# Autodesk Inventor assembly: Motor Driver V1.4
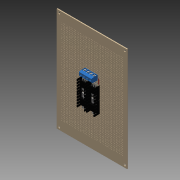
[picture p0: Inventor's stored thumbnail of the model, 180x180]
Saved by Autodesk Inventor 2015 (Build 190159000, 159)
## iProperties
Created: 2016-01-20
Part Number: Motor Driver V1.4
Document SubType Name: Assembly
Designer: Kyle
Author: Kyle
## Documents named in this file (18)
- C:\Users\Kyle\Documents\Project documentation\Motor driver\V1.4\CAD\Motor Driver V1.4.iam
- C:\Users\Kyle\Documents\Project documentation\Motor driver\V1.4\CAD\40x55 PC Board.ipt
- C:\Users\Kyle\Documents\Project documentation\Motor driver\V1.4\CAD\TO-220 Heatsink.ipt
- C:\Users\Kyle\Documents\Project documentation\Motor driver\V1.4\CAD\TO-220 Thermal Film.ipt
- C:\Users\Kyle\Documents\Project documentation\Motor driver\V1.4\CAD\TO-220 Transistor.iam
- C:\Users\Kyle\Documents\Project documentation\Motor driver\V1.4\CAD\6-32 14'' Screw.ipt
- C:\Users\Kyle\Documents\Project documentation\Motor driver\V1.4\CAD\6-32 Nut.ipt
- C:\Users\Kyle\Documents\Project documentation\Motor driver\V1.4\CAD\s470 Resistor.ipt
- C:\Users\Kyle\Documents\Project documentation\Motor driver\V1.4\CAD\Solder Joint.ipt
- C:\Users\Kyle\Documents\Project documentation\Motor driver\V1.4\CAD\sTLP152 Optocoupler.ipt
- C:\Users\Kyle\Documents\Project documentation\Motor driver\V1.4\CAD\s1k Resistor.ipt
- C:\Users\Kyle\Documents\Project documentation\Motor driver\V1.4\CAD\74LVC2G14 Dual Inverter.ipt
- C:\Users\Kyle\Documents\Project documentation\Motor driver\V1.4\CAD\s174 Resistor.ipt
- C:\Users\Kyle\Documents\Project documentation\Motor driver\V1.4\CAD\s74LVC2G08 Dual AND.ipt
- C:\Users\Kyle\Documents\Project documentation\Motor driver\V1.4\CAD\1x2 Terminal Block.iam
- C:\Users\Kyle\Documents\Project documentation\Motor driver\V1.4\CAD\s1uF Capacitor.ipt
- C:\Users\Kyle\Documents\Project documentation\Motor driver\V1.4\CAD\s20A 60V Diode.ipt
- C:\Users\Kyle\Documents\Project documentation\Motor driver\V1.4\CAD\Wire 3.ipt
## Components (95 placed, 17 different names)
1. 40x55 PC Board:1 — Mate:1, Mate:2, Mate:3, Mate:4, Mate:5, Angle:1, Mate:6, Angle:2, Angle:3, Mate:7, Mate:8, Mate:18, Mate:19, Mate:21, Mate:22, Mate:24, Mate:25, Mate:27, Mate:28, Mate:29, Mate:31, Mate:33, Mate:35, Mate:37, Mate:39, Mate:41, Mate:43, Mate:45, Angle:8, Mate:46, Mate:47, Mate:48, Mate:49, Angle:9, Mate:50, Mate:51, Mate:52, Mate:53, Mate:55, Mate:56, Mate:58, Mate:59, Mate:61, Mate:62, Mate:64, Mate:65, Mate:67, Mate:68, Mate:70, Mate:71, Mate:73, Mate:74, Mate:75, Mate:76, Mate:77, Mate:79, Mate:80, Mate:83, Mate:86, Mate:91, Mate:92, Mate:95, Mate:99, Mate:101, Mate:102, Mate:103, Mate:105, Mate:106, Angle:10, Flush:4, Mate:107, Mate:108, Mate:109, Flush:5, Mate:110, Mate:112, Mate:113, Flush:6, Flush:7, Flush:8, Flush:9, Mate:115, Mate:116, Mate:117, Mate:118, Mate:119, Mate:120, Flush:10, Flush:11, Flush:12, Flush:13, Mate:121, Mate:122, Mate:123, Mate:125, Mate:126, Mate:127, Mate:129, Mate:130, Mate:131, Mate:133, Mate:134, Mate:135, Mate:136, Mate:137, Mate:138, Mate:139, Mate:141, Mate:142, Mate:144, Mate:145, Mate:146, Mate:147, Mate:148, Mate:154, Mate:155, Mate:156, Mate:157, Flush:14, Flush:15, Mate:160, Mate:161, Mate:162, Mate:163, Mate:164, Mate:165, Mate:166, Mate:168, Mate:170, Mate:172, Mate:174, Mate:176, Mate:178, Mate:180, Mate:181, Mate:182, Mate:183, Mate:184, Mate:187, Mate:188, Mate:189, Mate:191, Angle:11, Mate:192, Mate:193, Mate:194, Angle:12, Angle:13, Flush:19, Flush:20, Flush:21, Mate:207, Angle:14, Mate:208, Mate:209, Mate:211, Mate:212, Mate:213, Mate:215, Mate:217, Mate:219, Mate:220, Mate:221, Mate:222, Mate:223, Mate:224, Mate:225, Mate:226, Mate:227, Mate:230, Mate:231, Mate:232, Mate:233, Mate:234, Mate:235, Mate:236, Mate:237, Mate:238, Mate:239, Mate:240, Angle:15, Tangent:1, Mate:241, Mate:242, Mate:243, Mate:244, Mate:245, Mate:247, Mate:251, Mate:252, Mate:253, Mate:254, Mate:255, Mate:256, Mate:257, Mate:259, Mate:261, Mate:263, Mate:265, Mate:267, Mate:269
2. TO-220 Heatsink:1 — Mate:1, Angle:3, Flush:3, Mate:7, Mate:9, Mate:10, Angle:4
3. TO-220 Heatsink:2 — Mate:3, Flush:1, Mate:6, Flush:2, Mate:13, Mate:14, Angle:6
4. TO-220 Heatsink:3 — Mate:2, Angle:2, Flush:2, Mate:8, Mate:15, Mate:16, Angle:7
5. TO-220 Heatsink:4 — Mate:4, Mate:5, Flush:1, Angle:1, Flush:3, Mate:11, Angle:5, Mate:12
6. TO-220 Thermal Film:1 — Mate:13, Mate:14, Angle:6, Mate:23
7. TO-220 Thermal Film:2 — Mate:15, Mate:16, Angle:7, Mate:26
8. TO-220 Thermal Film:3 — Mate:9, Mate:10, Angle:4, Mate:20
9. TO-220 Thermal Film:4 — Mate:11, Angle:5, Mate:12, Mate:17
10. TO-220 Transistor:1 [sub-assembly] — Mate:23, Mate:24, Mate:25, Mate:34
11. TO-220 Transistor:2 [sub-assembly] — Mate:26, Mate:27, Mate:28, Mate:30
12. TO-220 Transistor:3 [sub-assembly] — Mate:20, Mate:21, Mate:22, Mate:32
13. TO-220 Transistor:4 [sub-assembly] — Mate:17, Mate:18, Mate:19, Mate:36
14. 6-32 14'' Screw:1 — Mate:29, Mate:30, Mate:42
15. 6-32 14'' Screw:2 — Mate:31, Mate:32, Mate:38
16. 6-32 14'' Screw:3 — Mate:33, Mate:34, Mate:44
17. 6-32 14'' Screw:4 — Mate:35, Mate:36, Mate:40
18. 6-32 Nut:1 — Mate:37, Mate:38
19. 6-32 Nut:2 — Mate:39, Mate:40
20. 6-32 Nut:3 — Mate:41, Mate:42
21. 6-32 Nut:4 — Mate:43, Mate:44
22. s470 Resistor:1 — Mate:45, Angle:8, Mate:46, Mate:47
23. s470 Resistor:2 — Mate:48, Mate:49, Angle:9, Mate:50
24. Solder Joint:1 — Mate:72, Mate:73, Mate:74, Mate:111
25. Solder Joint:2 — Mate:69, Mate:70, Mate:71, Mate:72
26. Solder Joint:3 — Mate:63, Mate:64, Mate:65, Mate:66
27. Solder Joint:4 — Mate:51, Mate:52, Mate:53, Mate:54
28. Solder Joint:5 — Mate:54, Mate:55, Mate:56, Mate:57
29. Solder Joint:6 — Mate:60, Mate:61, Mate:62, Mate:63
30. Solder Joint:7 — Mate:57, Mate:58, Mate:59, Mate:60
31. Solder Joint:8 — Mate:66, Mate:67, Mate:68, Mate:69
32. Solder Joint:9 — Mate:75, Mate:76, Mate:77, Mate:78
33. Solder Joint:10 — Mate:78, Mate:79, Mate:80, Mate:81
34. Solder Joint:11 — Mate:81, Mate:83, Mate:99, Mate:100
35. Solder Joint:12 — Mate:86, Mate:100, Mate:101
36. Solder Joint:14 — Mate:95, Mate:102, Mate:103, Mate:104
37. Solder Joint:15 — Mate:91, Mate:92, Mate:104, Mate:114
38. sTLP152 Optocoupler:1 — Mate:106, Flush:6, Flush:7
39. sTLP152 Optocoupler:2 — Mate:105, Angle:10, Flush:4, Mate:107
40. s1k Resistor:1 — Mate:108, Mate:109, Flush:5
41. s1k Resistor:2 — Mate:113, Flush:8, Flush:9
42. Solder Joint:16 — Mate:110, Mate:111, Mate:112
43. Solder Joint:17 — Mate:114, Mate:115, Mate:116
44. 74LVC2G14 Dual Inverter:1 — Mate:117
45. s174 Resistor:1 — Mate:119, Flush:12, Flush:13
46. s174 Resistor:2 — Mate:118, Flush:10, Flush:11
47. s74LVC2G08 Dual AND:1 — Mate:120, Flush:14, Flush:15
48. Solder Joint:18 — Mate:121, Mate:122, Mate:123, Mate:124
49. Solder Joint:19 — Mate:124, Mate:125, Mate:126, Mate:128
50. Solder Joint:20 — Mate:127, Mate:128, Mate:129, Mate:132, Mate:167
51. Solder Joint:21 — Mate:130, Mate:131, Mate:132, Mate:150
52. Solder Joint:22 — Mate:133, Mate:134, Mate:135
53. Solder Joint:23 — Mate:136, Mate:137, Mate:138, Mate:140
54. Solder Joint:24 — Mate:139, Mate:140, Mate:141, Mate:143, Mate:185
55. Solder Joint:25 — Mate:142, Mate:143, Mate:144, Mate:159
56. Solder Joint:27 — Mate:148, Mate:149, Mate:150
57. Solder Joint:28 — Mate:145, Mate:146, Mate:147, Mate:149
58. Solder Joint:30 — Mate:157, Mate:158, Mate:159
59. Solder Joint:31 — Mate:154, Mate:155, Mate:156, Mate:158
60. Solder Joint:32 — Mate:160, Mate:167, Mate:168, Mate:169
61. Solder Joint:33 — Mate:161, Mate:169, Mate:170, Mate:171
62. Solder Joint:34 — Mate:162, Mate:171, Mate:172, Mate:173
63. Solder Joint:35 — Mate:163, Mate:173, Mate:174, Mate:175
64. Solder Joint:36 — Mate:164, Mate:175, Mate:176, Mate:177
65. Solder Joint:37 — Mate:165, Mate:177, Mate:178, Mate:179
66. Solder Joint:38 — Mate:166, Mate:179, Mate:180
67. Solder Joint:39 — Mate:181, Mate:184, Mate:185, Mate:186
68. Solder Joint:40 — Mate:182, Mate:186, Mate:187
69. Solder Joint:41 — Mate:183, Mate:188, Mate:189, Mate:210
70. 1x2 Terminal Block:1 [sub-assembly] — Mate:190, Flush:16, Flush:17, Angle:11, Mate:192, Mate:214, Mate:228
71. 1x2 Terminal Block:2 [sub-assembly] — Mate:190, Flush:16, Flush:17, Mate:191, Mate:246, Mate:258
72. s1uF Capacitor:1 — Mate:193, Angle:12, Flush:18, Flush:19, Flush:20
73. s1uF Capacitor:2 — Mate:194, Angle:13, Flush:18, Flush:21
74. s20A 60V Diode:1 — Mate:207, Angle:14
75. Solder Joint:42 — Mate:208, Mate:209, Mate:210
76. Solder Joint:43 — Mate:211, Mate:214, Mate:215, Mate:216
77. Solder Joint:44 — Mate:212, Mate:218, Mate:219
78. Solder Joint:45 — Mate:213, Mate:216, Mate:217, Mate:218
79. Solder Joint:46 — Mate:220, Mate:227, Mate:228, Mate:229
80. Solder Joint:47 — Mate:221, Mate:229, Mate:230, Mate:232
81. Solder Joint:48 — Mate:222, Mate:231, Mate:234
82. Solder Joint:49 — Mate:223, Mate:233, Mate:236
83. Solder Joint:50 — Mate:224, Mate:235, Mate:238
84. Solder Joint:51 — Mate:225, Mate:237
85. Solder Joint:52 — Mate:226, Mate:239, Mate:240
86. Wire 3:1 — Angle:15, Tangent:1, Mate:241, Mate:242, Mate:249, Mate:250
87. Solder Joint:53 — Mate:243, Mate:246, Mate:247, Mate:248
88. Solder Joint:54 — Mate:244, Mate:248, Mate:249
89. Solder Joint:55 — Mate:245, Mate:250, Mate:251
90. Solder Joint:56 — Mate:252, Mate:258, Mate:259, Mate:260
91. Solder Joint:57 — Mate:253, Mate:260, Mate:261, Mate:262
92. Solder Joint:58 — Mate:254, Mate:262, Mate:263, Mate:264
93. Solder Joint:59 — Mate:255, Mate:264, Mate:265, Mate:266
94. Solder Joint:60 — Mate:256, Mate:266, Mate:267, Mate:268
95. Solder Joint:61 — Mate:257, Mate:268, Mate:269
## Relationships (279: Mate 242, Flush 21, Angle 15, Tangent 1)
- Mate:1: 40x55 PC Board:1 ↔ TO-220 Heatsink:1
- Mate:2: 40x55 PC Board:1 ↔ TO-220 Heatsink:3
- Mate:3: 40x55 PC Board:1 ↔ TO-220 Heatsink:2
- Mate:4: 40x55 PC Board:1 ↔ TO-220 Heatsink:4
- Mate:5: 40x55 PC Board:1 ↔ TO-220 Heatsink:4
- Flush:1: TO-220 Heatsink:2 ↔ TO-220 Heatsink:4
- Angle:1 (0 deg): 40x55 PC Board:1 ↔ TO-220 Heatsink:4
- Mate:6: 40x55 PC Board:1 ↔ TO-220 Heatsink:2
- Angle:2 (0 deg): 40x55 PC Board:1 ↔ TO-220 Heatsink:3
- Angle:3 (0 deg): 40x55 PC Board:1 ↔ TO-220 Heatsink:1
- Flush:2: TO-220 Heatsink:2 ↔ TO-220 Heatsink:3
- Flush:3: TO-220 Heatsink:1 ↔ TO-220 Heatsink:4
- Mate:7: 40x55 PC Board:1 ↔ TO-220 Heatsink:1
- Mate:8: 40x55 PC Board:1 ↔ TO-220 Heatsink:3
- Mate:9: TO-220 Heatsink:1 ↔ TO-220 Thermal Film:3
- Mate:10: TO-220 Heatsink:1 ↔ TO-220 Thermal Film:3
- Angle:4 (0 deg): TO-220 Heatsink:1 ↔ TO-220 Thermal Film:3
- Mate:11: TO-220 Heatsink:4 ↔ TO-220 Thermal Film:4
- Angle:5 (0 deg): TO-220 Heatsink:4 ↔ TO-220 Thermal Film:4
- Mate:12: TO-220 Heatsink:4 ↔ TO-220 Thermal Film:4
- Mate:13: TO-220 Heatsink:2 ↔ TO-220 Thermal Film:1
- Mate:14: TO-220 Heatsink:2 ↔ TO-220 Thermal Film:1
- Angle:6 (0 deg): TO-220 Heatsink:2 ↔ TO-220 Thermal Film:1
- Mate:15: TO-220 Heatsink:3 ↔ TO-220 Thermal Film:2
- Mate:16: TO-220 Heatsink:3 ↔ TO-220 Thermal Film:2
- Angle:7 (0 deg): TO-220 Heatsink:3 ↔ TO-220 Thermal Film:2
- Mate:17: TO-220 Thermal Film:4 ↔ TO-220 Transistor:4
- Mate:18: 40x55 PC Board:1 ↔ TO-220 Transistor:4
- Mate:19: 40x55 PC Board:1 ↔ TO-220 Transistor:4
- Mate:20: TO-220 Thermal Film:3 ↔ TO-220 Transistor:3
- Mate:21: 40x55 PC Board:1 ↔ TO-220 Transistor:3
- Mate:22: 40x55 PC Board:1 ↔ TO-220 Transistor:3
- Mate:23: TO-220 Thermal Film:1 ↔ TO-220 Transistor:1
- Mate:24: 40x55 PC Board:1 ↔ TO-220 Transistor:1
- Mate:25: 40x55 PC Board:1 ↔ TO-220 Transistor:1
- Mate:26: TO-220 Thermal Film:2 ↔ TO-220 Transistor:2
- Mate:27: 40x55 PC Board:1 ↔ TO-220 Transistor:2
- Mate:28: 40x55 PC Board:1 ↔ TO-220 Transistor:2
- Mate:29: 40x55 PC Board:1 ↔ 6-32 14'' Screw:1
- Mate:30: TO-220 Transistor:2 ↔ 6-32 14'' Screw:1
- Mate:31: 40x55 PC Board:1 ↔ 6-32 14'' Screw:2
- Mate:32: TO-220 Transistor:3 ↔ 6-32 14'' Screw:2
- Mate:33: 40x55 PC Board:1 ↔ 6-32 14'' Screw:3
- Mate:34: TO-220 Transistor:1 ↔ 6-32 14'' Screw:3
- Mate:35: 40x55 PC Board:1 ↔ 6-32 14'' Screw:4
- Mate:36: TO-220 Transistor:4 ↔ 6-32 14'' Screw:4
- Mate:37: 40x55 PC Board:1 ↔ 6-32 Nut:1
- Mate:38: 6-32 14'' Screw:2 ↔ 6-32 Nut:1
- Mate:39: 40x55 PC Board:1 ↔ 6-32 Nut:2
- Mate:40: 6-32 14'' Screw:4 ↔ 6-32 Nut:2
- Mate:41: 40x55 PC Board:1 ↔ 6-32 Nut:3
- Mate:42: 6-32 14'' Screw:1 ↔ 6-32 Nut:3
- Mate:43: 40x55 PC Board:1 ↔ 6-32 Nut:4
- Mate:44: 6-32 14'' Screw:3 ↔ 6-32 Nut:4
- Mate:45: 40x55 PC Board:1 ↔ s470 Resistor:1
- Angle:8 (0 deg): 40x55 PC Board:1 ↔ s470 Resistor:1
- Mate:46 (1.016 mm): 40x55 PC Board:1 ↔ s470 Resistor:1
- Mate:47 (1.778 mm): 40x55 PC Board:1 ↔ s470 Resistor:1
- Mate:48: 40x55 PC Board:1 ↔ s470 Resistor:2
- Mate:49 (1.016 mm): 40x55 PC Board:1 ↔ s470 Resistor:2
- Angle:9 (0 deg): 40x55 PC Board:1 ↔ s470 Resistor:2
- Mate:50 (1.778 mm): 40x55 PC Board:1 ↔ s470 Resistor:2
- Mate:51: 40x55 PC Board:1 ↔ Solder Joint:4
- Mate:52: 40x55 PC Board:1 ↔ Solder Joint:4
- Mate:53: 40x55 PC Board:1 ↔ Solder Joint:4
- Mate:54: Solder Joint:4 ↔ Solder Joint:5
- Mate:55: 40x55 PC Board:1 ↔ Solder Joint:5
- Mate:56: 40x55 PC Board:1 ↔ Solder Joint:5
- Mate:57: Solder Joint:5 ↔ Solder Joint:7
- Mate:58: 40x55 PC Board:1 ↔ Solder Joint:7
- Mate:59: 40x55 PC Board:1 ↔ Solder Joint:7
- Mate:60: Solder Joint:6 ↔ Solder Joint:7
- Mate:61: 40x55 PC Board:1 ↔ Solder Joint:6
- Mate:62: 40x55 PC Board:1 ↔ Solder Joint:6
- Mate:63: Solder Joint:3 ↔ Solder Joint:6
- Mate:64: 40x55 PC Board:1 ↔ Solder Joint:3
- Mate:65: 40x55 PC Board:1 ↔ Solder Joint:3
- Mate:66: Solder Joint:3 ↔ Solder Joint:8
- Mate:67: 40x55 PC Board:1 ↔ Solder Joint:8
- Mate:68: 40x55 PC Board:1 ↔ Solder Joint:8
- Mate:69: Solder Joint:2 ↔ Solder Joint:8
- Mate:70: 40x55 PC Board:1 ↔ Solder Joint:2
- Mate:71: 40x55 PC Board:1 ↔ Solder Joint:2
- Mate:72: Solder Joint:1 ↔ Solder Joint:2
- Mate:73: 40x55 PC Board:1 ↔ Solder Joint:1
- Mate:74: 40x55 PC Board:1 ↔ Solder Joint:1
- Mate:75: 40x55 PC Board:1 ↔ Solder Joint:9
- Mate:76: 40x55 PC Board:1 ↔ Solder Joint:9
- Mate:77: 40x55 PC Board:1 ↔ Solder Joint:9
- Mate:78: Solder Joint:9 ↔ Solder Joint:10
- Mate:79: 40x55 PC Board:1 ↔ Solder Joint:10
- Mate:80: 40x55 PC Board:1 ↔ Solder Joint:10
- Mate:81: Solder Joint:10 ↔ Solder Joint:11
- Mate:83: 40x55 PC Board:1 ↔ Solder Joint:11
- Mate:86: 40x55 PC Board:1 ↔ Solder Joint:12
- Mate:91: 40x55 PC Board:1 ↔ Solder Joint:15
- Mate:92: 40x55 PC Board:1 ↔ Solder Joint:15
- Mate:95: 40x55 PC Board:1 ↔ Solder Joint:14
- Mate:99: 40x55 PC Board:1 ↔ Solder Joint:11
- Mate:100: Solder Joint:11 ↔ Solder Joint:12
- Mate:101: 40x55 PC Board:1 ↔ Solder Joint:12
- Mate:102: 40x55 PC Board:1 ↔ Solder Joint:14
- Mate:103: 40x55 PC Board:1 ↔ Solder Joint:14
- Mate:104: Solder Joint:14 ↔ Solder Joint:15
- Mate:105: 40x55 PC Board:1 ↔ sTLP152 Optocoupler:2
- Mate:106: 40x55 PC Board:1 ↔ sTLP152 Optocoupler:1
- Angle:10 (0 deg): 40x55 PC Board:1 ↔ sTLP152 Optocoupler:2
- Flush:4 (51.2572 mm): 40x55 PC Board:1 ↔ sTLP152 Optocoupler:2
- Mate:107 (0.508 mm): 40x55 PC Board:1 ↔ sTLP152 Optocoupler:2
- Mate:108: 40x55 PC Board:1 ↔ s1k Resistor:1
- Mate:109 (0.381 mm): 40x55 PC Board:1 ↔ s1k Resistor:1
- Flush:5 (49.911 mm): 40x55 PC Board:1 ↔ s1k Resistor:1
- Mate:110: 40x55 PC Board:1 ↔ Solder Joint:16
- Mate:111: Solder Joint:1 ↔ Solder Joint:16
- Mate:112: 40x55 PC Board:1 ↔ Solder Joint:16
- Mate:113: 40x55 PC Board:1 ↔ s1k Resistor:2
- Flush:6 (49.276 mm): 40x55 PC Board:1 ↔ sTLP152 Optocoupler:1
- Flush:7 (105.41 mm): 40x55 PC Board:1 ↔ sTLP152 Optocoupler:1
- Flush:8 (47.879 mm): 40x55 PC Board:1 ↔ s1k Resistor:2
- Flush:9 (111.252 mm): 40x55 PC Board:1 ↔ s1k Resistor:2
- Mate:114: Solder Joint:15 ↔ Solder Joint:17
- Mate:115: 40x55 PC Board:1 ↔ Solder Joint:17
- Mate:116: 40x55 PC Board:1 ↔ Solder Joint:17
- Mate:117: 40x55 PC Board:1 ↔ 74LVC2G14 Dual Inverter:1
- Mate:118: 40x55 PC Board:1 ↔ s174 Resistor:2
- Mate:119: 40x55 PC Board:1 ↔ s174 Resistor:1
- Mate:120: 40x55 PC Board:1 ↔ s74LVC2G08 Dual AND:1
- Flush:10 (81.026 mm): 40x55 PC Board:1 ↔ s174 Resistor:2
- Flush:11 (54.864 mm): 40x55 PC Board:1 ↔ s174 Resistor:2
- Flush:12 (59.944 mm): 40x55 PC Board:1 ↔ s174 Resistor:1
- Flush:13 (63.881 mm): 40x55 PC Board:1 ↔ s174 Resistor:1
- Mate:121: 40x55 PC Board:1 ↔ Solder Joint:18
- Mate:122: 40x55 PC Board:1 ↔ Solder Joint:18
- Mate:123: 40x55 PC Board:1 ↔ Solder Joint:18
- Mate:124: Solder Joint:18 ↔ Solder Joint:19
- Mate:125: 40x55 PC Board:1 ↔ Solder Joint:19
- Mate:126: 40x55 PC Board:1 ↔ Solder Joint:19
- Mate:127: 40x55 PC Board:1 ↔ Solder Joint:20
- Mate:128: Solder Joint:19 ↔ Solder Joint:20
- Mate:129: 40x55 PC Board:1 ↔ Solder Joint:20
- Mate:130: 40x55 PC Board:1 ↔ Solder Joint:21
- Mate:131: 40x55 PC Board:1 ↔ Solder Joint:21
- Mate:132: Solder Joint:20 ↔ Solder Joint:21
- Mate:133: 40x55 PC Board:1 ↔ Solder Joint:22
- Mate:134: 40x55 PC Board:1 ↔ Solder Joint:22
- Mate:135: 40x55 PC Board:1 ↔ Solder Joint:22
- Mate:136: 40x55 PC Board:1 ↔ Solder Joint:23
- Mate:137: 40x55 PC Board:1 ↔ Solder Joint:23
- Mate:138: 40x55 PC Board:1 ↔ Solder Joint:23
- Mate:139: 40x55 PC Board:1 ↔ Solder Joint:24
- Mate:140: Solder Joint:23 ↔ Solder Joint:24
- Mate:141: 40x55 PC Board:1 ↔ Solder Joint:24
- Mate:142: 40x55 PC Board:1 ↔ Solder Joint:25
- Mate:143: Solder Joint:24 ↔ Solder Joint:25
- Mate:144: 40x55 PC Board:1 ↔ Solder Joint:25
- Mate:145: 40x55 PC Board:1 ↔ Solder Joint:28
- Mate:146: 40x55 PC Board:1 ↔ Solder Joint:28
- Mate:147: 40x55 PC Board:1 ↔ Solder Joint:28
- Mate:148: 40x55 PC Board:1 ↔ Solder Joint:27
- Mate:149: Solder Joint:27 ↔ Solder Joint:28
- Mate:150: Solder Joint:21 ↔ Solder Joint:27
- Mate:154: 40x55 PC Board:1 ↔ Solder Joint:31
- Mate:155: 40x55 PC Board:1 ↔ Solder Joint:31
- Mate:156: 40x55 PC Board:1 ↔ Solder Joint:31
- Mate:157: 40x55 PC Board:1 ↔ Solder Joint:30
- Mate:158: Solder Joint:30 ↔ Solder Joint:31
- Mate:159: Solder Joint:25 ↔ Solder Joint:30
- Flush:14 (54.61 mm): 40x55 PC Board:1 ↔ s74LVC2G08 Dual AND:1
- Flush:15 (91.186 mm): 40x55 PC Board:1 ↔ s74LVC2G08 Dual AND:1
- Mate:160: 40x55 PC Board:1 ↔ Solder Joint:32
- Mate:161: 40x55 PC Board:1 ↔ Solder Joint:33
- Mate:162: 40x55 PC Board:1 ↔ Solder Joint:34
- Mate:163: 40x55 PC Board:1 ↔ Solder Joint:35
- Mate:164: 40x55 PC Board:1 ↔ Solder Joint:36
- Mate:165: 40x55 PC Board:1 ↔ Solder Joint:37
- Mate:166: 40x55 PC Board:1 ↔ Solder Joint:38
- Mate:167: Solder Joint:20 ↔ Solder Joint:32
- Mate:168: 40x55 PC Board:1 ↔ Solder Joint:32
- Mate:169: Solder Joint:32 ↔ Solder Joint:33
- Mate:170: 40x55 PC Board:1 ↔ Solder Joint:33
- Mate:171: Solder Joint:33 ↔ Solder Joint:34
- Mate:172: 40x55 PC Board:1 ↔ Solder Joint:34
- Mate:173: Solder Joint:34 ↔ Solder Joint:35
- Mate:174: 40x55 PC Board:1 ↔ Solder Joint:35
- Mate:175: Solder Joint:35 ↔ Solder Joint:36
- Mate:176: 40x55 PC Board:1 ↔ Solder Joint:36
- Mate:177: Solder Joint:36 ↔ Solder Joint:37
- Mate:178: 40x55 PC Board:1 ↔ Solder Joint:37
- Mate:179: Solder Joint:37 ↔ Solder Joint:38
- Mate:180: 40x55 PC Board:1 ↔ Solder Joint:38
- Mate:181: 40x55 PC Board:1 ↔ Solder Joint:39
- Mate:182: 40x55 PC Board:1 ↔ Solder Joint:40
- Mate:183: 40x55 PC Board:1 ↔ Solder Joint:41
- Mate:184: 40x55 PC Board:1 ↔ Solder Joint:39
- Mate:185: Solder Joint:24 ↔ Solder Joint:39
- Mate:186: Solder Joint:39 ↔ Solder Joint:40
- Mate:187: 40x55 PC Board:1 ↔ Solder Joint:40
- Mate:188: 40x55 PC Board:1 ↔ Solder Joint:41
- Mate:189: 40x55 PC Board:1 ↔ Solder Joint:41
- Mate:190: 1x2 Terminal Block:1 ↔ 1x2 Terminal Block:2
- Flush:16: 1x2 Terminal Block:1 ↔ 1x2 Terminal Block:2
- Flush:17: 1x2 Terminal Block:1 ↔ 1x2 Terminal Block:2
- Mate:191: 40x55 PC Board:1 ↔ 1x2 Terminal Block:2
- Angle:11 (0 deg): 40x55 PC Board:1 ↔ 1x2 Terminal Block:1
- Mate:192: 40x55 PC Board:1 ↔ 1x2 Terminal Block:1
- Mate:193: 40x55 PC Board:1 ↔ s1uF Capacitor:1
- Mate:194: 40x55 PC Board:1 ↔ s1uF Capacitor:2
- Angle:12 (0 deg): 40x55 PC Board:1 ↔ s1uF Capacitor:1
- Angle:13 (0 deg): 40x55 PC Board:1 ↔ s1uF Capacitor:2
- Flush:18: s1uF Capacitor:1 ↔ s1uF Capacitor:2
- Flush:19 (62.865 mm): 40x55 PC Board:1 ↔ s1uF Capacitor:1
- Flush:20 (52.07 mm): 40x55 PC Board:1 ↔ s1uF Capacitor:1
- Flush:21 (62.23 mm): 40x55 PC Board:1 ↔ s1uF Capacitor:2
- Mate:207: 40x55 PC Board:1 ↔ s20A 60V Diode:1
- Angle:14 (0 deg): 40x55 PC Board:1 ↔ s20A 60V Diode:1
- Mate:208: 40x55 PC Board:1 ↔ Solder Joint:42
- Mate:209: 40x55 PC Board:1 ↔ Solder Joint:42
- Mate:210: Solder Joint:41 ↔ Solder Joint:42
- Mate:211: 40x55 PC Board:1 ↔ Solder Joint:43
- Mate:212: 40x55 PC Board:1 ↔ Solder Joint:44
- Mate:213: 40x55 PC Board:1 ↔ Solder Joint:45
- Mate:214: 1x2 Terminal Block:1 ↔ Solder Joint:43
- Mate:215: 40x55 PC Board:1 ↔ Solder Joint:43
- Mate:216: Solder Joint:43 ↔ Solder Joint:45
- Mate:217: 40x55 PC Board:1 ↔ Solder Joint:45
- Mate:218: Solder Joint:44 ↔ Solder Joint:45
- Mate:219: 40x55 PC Board:1 ↔ Solder Joint:44
- Mate:220: 40x55 PC Board:1 ↔ Solder Joint:46
- Mate:221: 40x55 PC Board:1 ↔ Solder Joint:47
- Mate:222: 40x55 PC Board:1 ↔ Solder Joint:48
- Mate:223: 40x55 PC Board:1 ↔ Solder Joint:49
- Mate:224: 40x55 PC Board:1 ↔ Solder Joint:50
- Mate:225: 40x55 PC Board:1 ↔ Solder Joint:51
- Mate:226: 40x55 PC Board:1 ↔ Solder Joint:52
- Mate:227: 40x55 PC Board:1 ↔ Solder Joint:46
- Mate:228: 1x2 Terminal Block:1 ↔ Solder Joint:46
- Mate:229: Solder Joint:46 ↔ Solder Joint:47
- Mate:230: 40x55 PC Board:1 ↔ Solder Joint:47
- Mate:231: 40x55 PC Board:1 ↔ Solder Joint:48
- Mate:232: 40x55 PC Board:1 ↔ Solder Joint:47
- Mate:233: 40x55 PC Board:1 ↔ Solder Joint:49
- Mate:234: 40x55 PC Board:1 ↔ Solder Joint:48
- Mate:235: 40x55 PC Board:1 ↔ Solder Joint:50
- Mate:236: 40x55 PC Board:1 ↔ Solder Joint:49
- Mate:237: 40x55 PC Board:1 ↔ Solder Joint:51
- Mate:238: 40x55 PC Board:1 ↔ Solder Joint:50
- Mate:239: 40x55 PC Board:1 ↔ Solder Joint:52
- Mate:240: 40x55 PC Board:1 ↔ Solder Joint:52
- Angle:15 (180 deg): 40x55 PC Board:1 ↔ Wire 3:1
- Tangent:1: 40x55 PC Board:1 ↔ Wire 3:1
- Mate:241: 40x55 PC Board:1 ↔ Wire 3:1
- Mate:242: 40x55 PC Board:1 ↔ Wire 3:1
- Mate:243: 40x55 PC Board:1 ↔ Solder Joint:53
- Mate:244: 40x55 PC Board:1 ↔ Solder Joint:54
- Mate:245: 40x55 PC Board:1 ↔ Solder Joint:55
- Mate:246: 1x2 Terminal Block:2 ↔ Solder Joint:53
- Mate:247: 40x55 PC Board:1 ↔ Solder Joint:53
- Mate:248: Solder Joint:53 ↔ Solder Joint:54
- Mate:249: Wire 3:1 ↔ Solder Joint:54
- Mate:250: Wire 3:1 ↔ Solder Joint:55
- Mate:251: 40x55 PC Board:1 ↔ Solder Joint:55
- Mate:252: 40x55 PC Board:1 ↔ Solder Joint:56
- Mate:253: 40x55 PC Board:1 ↔ Solder Joint:57
- Mate:254: 40x55 PC Board:1 ↔ Solder Joint:58
- Mate:255: 40x55 PC Board:1 ↔ Solder Joint:59
- Mate:256: 40x55 PC Board:1 ↔ Solder Joint:60
- Mate:257: 40x55 PC Board:1 ↔ Solder Joint:61
- Mate:258: 1x2 Terminal Block:2 ↔ Solder Joint:56
- Mate:259: 40x55 PC Board:1 ↔ Solder Joint:56
- Mate:260: Solder Joint:56 ↔ Solder Joint:57
- Mate:261: 40x55 PC Board:1 ↔ Solder Joint:57
- Mate:262: Solder Joint:57 ↔ Solder Joint:58
- Mate:263: 40x55 PC Board:1 ↔ Solder Joint:58
- Mate:264: Solder Joint:58 ↔ Solder Joint:59
- Mate:265: 40x55 PC Board:1 ↔ Solder Joint:59
- Mate:266: Solder Joint:59 ↔ Solder Joint:60
- Mate:267: 40x55 PC Board:1 ↔ Solder Joint:60
- Mate:268: Solder Joint:60 ↔ Solder Joint:61
- Mate:269: 40x55 PC Board:1 ↔ Solder Joint:61
